# Autodesk Inventor assembly: CollectorHolderAssembly
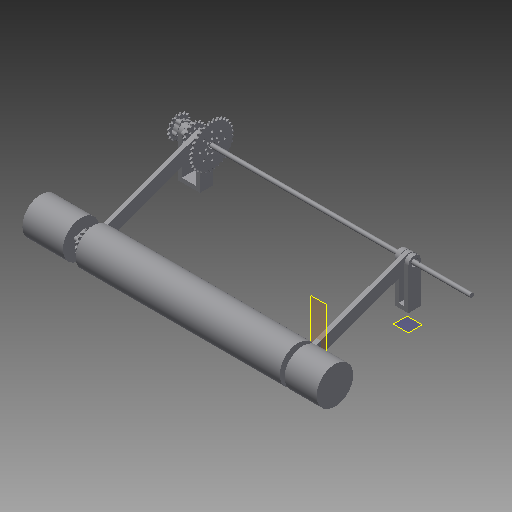
[picture p0: Inventor's stored thumbnail of the model, 512x512]
Saved by Autodesk Inventor 2017 (Build 210142000, 142)
## iProperties
Created: 2017-04-19
Part Number: CollectorHolderAssembly
Document SubType Name: Assembly
Designer: User
Author: User
## Documents named in this file (11)
- C:\Robotics\CAD\2016-17_CAD\Collector\CollectorHolderAssembly.iam
- C:\Robotics\CAD\2016-17_CAD\Collector\CollectorHolder.ipt
- C:\Robotics\CAD\2016-17_CAD\Custom COTS\Axle18in.ipt
- C:\Robotics\CAD\COTSParts\Actobotics\535 parts\535198Bearing.25ID.5OD.ipt
- C:\Robotics\CAD\COTSParts\Actobotics\545 parts\545556SetScrewHub.77inPattern.ipt
- C:\Robotics\CAD\COTSParts\Actobotics\615 parts\615102Sprocket.5inBore.25inPitch16Teeth.ipt
- C:\Robotics\CAD\2016-17_CAD\Collector\RollerArm.ipt
- C:\Robotics\CAD\2016-17_CAD\Collector\CollecterHolderShort.ipt
- C:\Robotics\CAD\2016-17_CAD\Custom COTS\Axle1.34.ipt
- C:\Robotics\CAD\2016-17_CAD\Collector\RollerFull.ipt
- C:\Robotics\CAD\COTSParts\Actobotics\615 parts\615114Sprocket.5inBore.25inPitch32Teeth.ipt
## Components (22 placed, 10 different names)
1. CollectorHolder:1 — Insert:1, Insert:2, Insert:3, Insert:4, Insert:5, Flush:1, Flush:2
2. Axle18in:1 — Insert:3
3. 535198Bearing.25ID.5OD:1 — Insert:1, Insert:6
4. 535198Bearing.25ID.5OD:2 — Insert:2, Insert:10
5. 545556SetScrewHub.77inPattern:1 — Insert:4, Insert:22
6. 545556SetScrewHub.77inPattern:2 — Insert:5, Insert:9
7. 545556SetScrewHub.77inPattern:3 — Insert:6, Insert:7
8. 615102Sprocket.5inBore.25inPitch16Teeth:1 — Insert:9
9. 615102Sprocket.5inBore.25inPitch16Teeth:3 — Insert:7
10. RollerArm:1 — Insert:10, Insert:16, Insert:17
11. CollecterHolderShort:1 — Insert:11, Insert:12, Insert:13, Flush:1, Flush:2, Flush:3, Flush:4
12. RollerArm:2 — Insert:14, Insert:15, Insert:20
13. 535198Bearing.25ID.5OD:3 — Insert:11, Insert:14
14. 535198Bearing.25ID.5OD:4 — Insert:12
15. Axle1.34:1 — Insert:13
16. Axle18in:1 — Insert:15, Insert:16, Insert:21
17. 535198Bearing.25ID.5OD:5 — Insert:17, Insert:18
18. 615102Sprocket.5inBore.25inPitch16Teeth:4 — Insert:18, Insert:19
19. 545556SetScrewHub.77inPattern:4 — Insert:19
20. 535198Bearing.25ID.5OD:6 — Insert:20
21. RollerFull:1 — Insert:21, Tangent:1
22. 615114Sprocket.5inBore.25inPitch32Teeth:1 — Insert:22
## Relationships (26: Insert 21, Flush 4, Tangent 1)
- Insert:1: CollectorHolder:1 ↔ 535198Bearing.25ID.5OD:1
- Insert:2: CollectorHolder:1 ↔ 535198Bearing.25ID.5OD:2
- Insert:3 (-9.779 mm): CollectorHolder:1 ↔ Axle18in:1
- Insert:4: CollectorHolder:1 ↔ 545556SetScrewHub.77inPattern:1
- Insert:5: CollectorHolder:1 ↔ 545556SetScrewHub.77inPattern:2
- Insert:6: 535198Bearing.25ID.5OD:1 ↔ 545556SetScrewHub.77inPattern:3
- Insert:7: 545556SetScrewHub.77inPattern:3 ↔ 615102Sprocket.5inBore.25inPitch16Teeth:3
- Insert:9: 545556SetScrewHub.77inPattern:2 ↔ 615102Sprocket.5inBore.25inPitch16Teeth:1
- Insert:10: 535198Bearing.25ID.5OD:2 ↔ RollerArm:1
- Insert:11: CollecterHolderShort:1 ↔ 535198Bearing.25ID.5OD:3
- Insert:12: CollecterHolderShort:1 ↔ 535198Bearing.25ID.5OD:4
- Insert:13 (-6.35 mm): CollecterHolderShort:1 ↔ Axle1.34:1
- Insert:14: RollerArm:2 ↔ 535198Bearing.25ID.5OD:3
- Flush:1: CollectorHolder:1 ↔ CollecterHolderShort:1
- Flush:2: CollectorHolder:1 ↔ CollecterHolderShort:1
- Insert:15 (-50.8 mm): RollerArm:2 ↔ Axle18in:1
- Insert:16 (76.2 mm): RollerArm:1 ↔ Axle18in:1
- Insert:17: RollerArm:1 ↔ 535198Bearing.25ID.5OD:5
- Insert:18 (2.667 mm): 535198Bearing.25ID.5OD:5 ↔ 615102Sprocket.5inBore.25inPitch16Teeth:4
- Insert:19: 615102Sprocket.5inBore.25inPitch16Teeth:4 ↔ 545556SetScrewHub.77inPattern:4
- Insert:20: RollerArm:2 ↔ 535198Bearing.25ID.5OD:6
- Insert:21: Axle18in:1 ↔ RollerFull:1
- Insert:22: 545556SetScrewHub.77inPattern:1 ↔ 615114Sprocket.5inBore.25inPitch32Teeth:1
- Flush:3 (25.4 mm): CollecterHolderShort:1
- Flush:4 (128.905 mm): CollecterHolderShort:1
- Tangent:1: RollerFull:1
